# Autodesk Inventor assembly: Сборка2
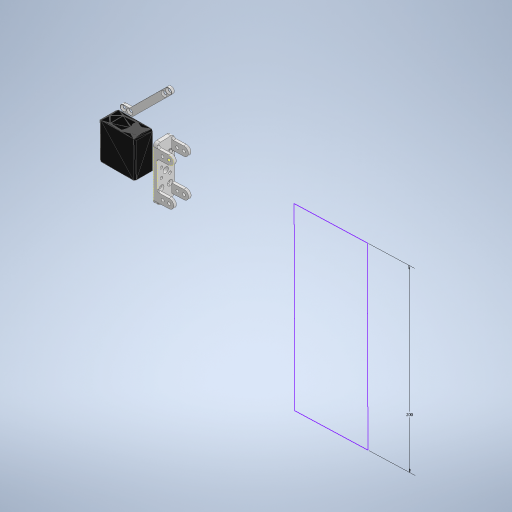
[picture p0: Inventor's stored thumbnail of the model, 512x512]
Saved by Autodesk Inventor 2023.1 (Build 271208000, 208)
## iProperties
Created: 2025-09-24
Part Number: Сборка2
Document SubType Name: Assembly
Designer: DELL
Author: DELL
## Documents named in this file (6)
- C:\Users\DELL\reposGitHub\Cheburashka\Cheburashka_construction\face\лицо\Сборка2.iam
- C:\Users\DELL\reposGitHub\Cheburashka\Cheburashka_construction\korpus\ds3240\emiliooros\servomotor-ds3240\Servo.ipt
- C:\Users\DELL\reposGitHub\Cheburashka\Cheburashka_construction\korpus\ds3240\emiliooros\servomotor-ds3240\acc2.ipt
- C:\Users\DELL\reposGitHub\Cheburashka\Cheburashka_construction\korpus\крепление_кракаса.ipt
- C:\Users\DELL\reposGitHub\Cheburashka\Cheburashka_construction\korpus\каркас1.ipt
- C:\Users\DELL\reposGitHub\Cheburashka\Cheburashka_construction\platform\legs\фанера_ухо.ipt
## Components (5 placed, 5 different names)
1. Servo:1 — Совмещение:1, Совмещение:2
2. acc2:1 — Совмещение:1, Совмещение:2, Совмещение:3, Угол:1
3. крепление_кракаса:1 — Заподлицо:1, Заподлицо:2, Заподлицо:3
4. каркас1:1
5. фанера_ухо:1 — Заподлицо:3
## Relationships (7: Mate 3, Flush 3, Angle 1)
- Совмещение:1 [Mate]: Servo:1 ↔ acc2:1
- Совмещение:2 [Mate]: Servo:1 ↔ acc2:1
- Совмещение:3 [Mate]: acc2:1
- Угол:1 [Angle] (0 deg): acc2:1
- Заподлицо:1 [Flush]: крепление_кракаса:1
- Заподлицо:2 [Flush]: крепление_кракаса:1
- Заподлицо:3 [Flush]: крепление_кракаса:1 ↔ фанера_ухо:1
